# Autodesk Inventor assembly: 球軸測試
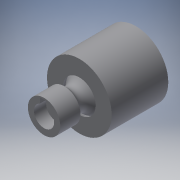
[picture p0: Inventor's stored thumbnail of the model, 180x180]
Saved by Autodesk Inventor 2017 (Build 210142000, 142)
## iProperties
Part Number: 球軸測試
Material: 一般
Document SubType Name: Assembly
Designer: NB23-1
Author: NB23-1
## Documents named in this file (3)
- C:\Users\NB23-1\Desktop\做爽的\迷你三軸平台\球軸測試.iam
- C:\Users\NB23-1\Desktop\做爽的\迷你三軸平台\伸縮缸 球軸 球.ipt
- C:\Users\NB23-1\Desktop\做爽的\迷你三軸平台\伸縮缸 球軸 座.ipt
## Components (2 placed, 2 different names)
1. 伸縮缸 球軸 球:1 — 貼合:1, 角度:1
2. 伸縮缸 球軸 座:1 — 貼合:1, 角度:1
## Relationships (2: Mate 1, Angle 1)
- 貼合:1 [Mate]: 伸縮缸 球軸 球:1 ↔ 伸縮缸 球軸 座:1
- 角度:1 [Angle] (0 deg): 伸縮缸 球軸 球:1 ↔ 伸縮缸 球軸 座:1
